# Autodesk Inventor assembly: Frame
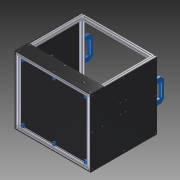
[picture p0: Inventor's stored thumbnail of the model, 180x180]
Saved by Autodesk Inventor 2015 SP1 (Build 190203100, 203)
## iProperties
Created: 2014-08-02
Part Number: Frame
Document SubType Name: Assembly
Designer: Jack
Mass: 9359.12 g
Surface Area: 35492.7 cm^2
Volume: 6557 cm^3
Density: 1.42735 g/cm^3
Author: Jack
Title: Frame
## Documents named in this file (25)
- C:\Users\Jack\ownCloud\Projects\CrossBot\InventorModel\Frame\Frame.iam
- C:\Users\Jack\ownCloud\Projects\CrossBot\InventorModel\Frame\FrameFrontBack.ipt
- C:\Users\Jack\ownCloud\Projects\CrossBot\InventorModel\Frame\FrameSide.ipt
- C:\Users\Jack\ownCloud\Projects\CrossBot\InventorModel\Frame\FrameUpright.ipt
- C:\Users\Jack\ownCloud\Projects\CrossBot\InventorModel\Hardware\Bolts\BlindExtrusionScrew\M5x20BlindScrew.ipt
- C:\Users\Jack\ownCloud\Projects\CrossBot\InventorModel\Frame\FrameExtruderVerticalSupport.ipt
- C:\Users\Jack\ownCloud\Projects\CrossBot\InventorModel\Enclosure\EnclosurePanelBack.ipt
- C:\Users\Jack\ownCloud\Projects\CrossBot\InventorModel\Enclosure\EnclosurePanelBottomFront.ipt
- C:\Users\Jack\ownCloud\Projects\CrossBot\InventorModel\Enclosure\ElectronicsLowerPanel.ipt
- C:\Users\Jack\ownCloud\Projects\CrossBot\InventorModel\Hardware\FrameBrace\FrameBraceHBLFSN5-4.ipt
- C:\Users\Jack\ownCloud\Projects\CrossBot\InventorModel\Enclosure\ElectronicsTopPanel.ipt
- C:\Users\Jack\ownCloud\Projects\CrossBot\InventorModel\Hardware\Bolts\SHCS\SHCS4\SHCS4x10.ipt
- C:\Users\Jack\ownCloud\Projects\CrossBot\InventorModel\Hardware\Nuts\ExtrusionNuts\ExtrusionNutLockHNTR5-4.ipt
- C:\Users\Jack\ownCloud\Projects\CrossBot\InventorModel\Hardware\Bolts\FHS\FHS4\FHS4x10.ipt
- C:\Users\Jack\ownCloud\Projects\CrossBot\InventorModel\Enclosure\EnclosurePanelLeft.ipt
- C:\Users\Jack\ownCloud\Projects\CrossBot\InventorModel\Enclosure\EnclosurePanelRight.ipt
- C:\Users\Jack\ownCloud\Projects\CrossBot\InventorModel\Enclosure\PanelMount.ipt
- C:\Users\Jack\ownCloud\Projects\CrossBot\InventorModel\Hardware\BoltWashers\BoltWasher3\BoltWasher3x18.iam
- C:\Users\Jack\ownCloud\Projects\CrossBot\InventorModel\Hardware\Nuts\Nut3.ipt
- C:\Users\Jack\ownCloud\Projects\CrossBot\InventorModel\Enclosure\PanelLedge.ipt
- C:\Users\Jack\ownCloud\Projects\CrossBot\InventorModel\Hardware\Nuts\ExtrusionNuts\ExtrusionNutHNKK5_4.ipt
- C:\Users\Jack\ownCloud\Projects\CrossBot\InventorModel\Enclosure\SpoolHolder\SpoolHolderSingle.ipt
- C:\Users\Jack\ownCloud\Projects\CrossBot\InventorModel\Hardware\Nuts\Nut4.ipt
- C:\Users\Jack\ownCloud\Projects\CrossBot\InventorModel\Enclosure\FrameHandle.ipt
- C:\Users\Jack\ownCloud\Projects\CrossBot\InventorModel\Hardware\Nuts\ExtrusionNuts\ExtrusionNutHNKK5_5.ipt
## Components (217 placed, 24 different names)
1. FrameSide:6 — Mate:66, Flush:32, Flush:33, Mate:136, Mate:181, Mate:183, Angle:21, Mate:328, Mate:460, Mate:498, Mate:500, Angle:62, Mate:513
2. FrameSide:5 — Mate:64, Flush:28, Flush:30, Mate:138, Mate:180, Mate:184, Angle:36, Angle:51, Mate:398, Mate:497, Mate:499, Angle:63, Mate:512
3. FrameSide:4 — Mate:52, Flush:23, Flush:25, Flush:26, Angle:35, Angle:50, Mate:397, Mate:437, Mate:438
4. FrameSide:3 — Mate:51, Flush:22, Flush:27, Angle:20, Mate:329, Mate:436, Mate:439, Mate:440
5. FrameSide:1 — Mate:1, Flush:1, Flush:2, Mate:3, Flush:5, Flush:6, Mate:18, Mate:22, Angle:25, Mate:342, Flush:114, Mate:363, Angle:95, Angle:96, Mate:616, Mate:617, Flush:165, Mate:618
6. FrameSide:2 — Mate:6, Flush:11, Flush:12, Mate:7, Mate:25, Mate:26, Mate:343, Flush:113, Angle:40, Mate:379, Angle:93, Mate:609, Mate:610, Flush:164, Angle:94, Mate:612
7. FrameExtruderVerticalSupport:1 — Mate:67, Flush:37, Mate:69, Mate:123, Flush:64, Mate:176, Mate:178, Mate:524, Angle:67
8. FrameExtruderVerticalSupport:2 — Mate:68, Flush:36, Mate:70, Mate:124, Flush:65, Mate:177, Mate:179, Mate:522, Angle:68
9. FrameUpright:1 — Mate:1, Flush:1, Flush:2, Mate:2, Flush:3, Flush:4, Mate:42, Mate:43, Mate:48, Mate:49, Mate:53, Flush:21, Flush:22, Mate:61, Mate:62, Mate:65, Mate:66, Flush:33, Flush:34, Mate:70, Flush:69, Mate:132, Mate:191, Mate:199, Angle:22, Angle:23, Angle:24, Mate:325, Mate:326, Mate:327, Angle:47, Angle:48, Angle:49, Mate:390, Mate:391, Mate:392, Mate:523, Angle:69
10. FrameUpright:2 — Mate:3, Flush:5, Flush:6, Mate:5, Flush:9, Flush:10, Mate:12, Mate:13, Mate:19, Mate:21, Mate:36, Mate:37, Mate:50, Mate:51, Mate:54, Mate:55, Mate:56, Flush:61, Mate:137, Flush:71, Mate:192, Mate:193, Mate:281, Angle:17, Angle:18, Mate:323, Angle:19, Mate:324, Angle:26, Angle:27, Mate:338, Mate:339, Flush:115, Mate:517, Angle:65
11. FrameUpright:3 — Mate:7, Mate:8, Flush:13, Mate:38, Mate:39, Mate:46, Mate:47, Mate:52, Flush:23, Flush:24, Mate:57, Mate:58, Mate:63, Mate:64, Flush:28, Flush:29, Mate:139, Flush:72, Mate:194, Mate:195, Angle:28, Angle:29, Mate:336, Mate:337, Flush:116, Mate:365, Angle:32, Mate:367, Mate:369, Angle:33, Angle:34, Mate:515, Angle:64
12. FrameUpright:4 — Mate:4, Flush:7, Flush:8, Mate:6, Flush:11, Flush:12, Mate:40, Mate:41, Mate:44, Mate:45, Mate:59, Mate:60, Mate:69, Mate:134, Flush:70, Mate:190, Mate:198, Mate:373, Angle:37, Mate:375, Angle:38, Mate:377, Angle:39, Flush:135, Mate:381, Angle:41, Angle:43, Angle:44, Mate:395, Mate:396, Mate:525, Angle:66
13. FrameFrontBack:3 — Mate:50, Flush:24, Flush:25, Mate:54, Flush:35, Flush:39, Angle:31, Mate:341, Mate:430, Mate:431, Mate:432, Angle:83, Angle:84, Angle:85, Mate:596, Mate:597, Mate:598, Mate:599
14. FrameFrontBack:6 — Mate:65, Flush:34, Mate:67, Mate:68, Flush:36, Flush:37, Mate:122, Mate:125, Mate:130, Mate:135, Mate:186, Mate:187, Mate:196, Mate:197, Angle:45, Mate:393, Mate:490, Mate:492, Angle:58, Mate:503, Mate:505, Angle:59, Angle:60, Angle:61, Mate:508, Mate:509, Angle:81, Angle:82, Mate:594, Mate:603
15. FrameFrontBack:5 — Mate:63, Flush:29, Flush:30, Flush:32, Flush:35, Mate:73, Mate:182, Mate:185, Angle:30, Mate:340, Mate:447, Flush:138, Mate:488, Mate:489, Angle:86, Angle:87, Angle:88, Mate:600, Mate:604
16. FrameFrontBack:4 — Mate:53, Flush:21, Flush:26, Flush:27, Flush:44, Angle:46, Mate:394, Mate:433, Mate:435, Mate:570, Flush:151, Angle:89, Angle:90, Angle:91, Mate:595, Mate:601, Mate:602
17. FrameFrontBack:1 — Mate:2, Flush:3, Flush:4, Mate:4, Flush:7, Flush:8, Mate:23, Mate:24, Mate:76, Mate:188, Mate:189, Angle:42, Mate:399
18. FrameFrontBack:2 — Mate:5, Flush:9, Flush:10, Mate:8, Flush:13, Flush:20, Mate:20, Mate:27
19. FrameHandle:1 — Mate:610, Flush:164, Mate:611, Mate:613
20. ExtrusionNutHNKK5_5:1 — Angle:93, Mate:609, Mate:611
21. ExtrusionNutHNKK5_5:2 — Angle:94, Mate:612, Mate:613
22. FrameHandle:2 — Flush:165, Mate:618
23. ExtrusionNutHNKK5_5:3 — Angle:95, Mate:616
24. ExtrusionNutHNKK5_5:4 — Angle:96, Mate:617
25. ExtrusionNutHNKK5_4:17 — Mate:583, Angle:89, Mate:602
26. ExtrusionNutHNKK5_4:18 — Mate:584, Angle:90, Mate:601
27. ExtrusionNutHNKK5_4:19 — Mate:585, Angle:91, Mate:595
28. ExtrusionNutHNKK5_4:20 — Mate:586, Angle:85, Mate:596
29. ExtrusionNutHNKK5_4:21 — Mate:587, Angle:84, Mate:598
30. ExtrusionNutHNKK5_4:22 — Mate:588, Angle:83, Mate:599
31. FHS4x10:43 — Mate:576, Flush:155, Mate:583
32. FHS4x10:47 — Mate:572, Flush:156, Mate:584
33. FHS4x10:46 — Mate:573, Flush:157, Mate:585
34. FHS4x10:51 — Mate:581, Flush:162, Mate:587
35. FHS4x10:52 — Mate:582, Flush:163, Mate:588
36. FHS4x10:50 — Mate:580, Flush:161, Mate:586
37. PanelLedge:6 — Mate:570, Flush:151, Mate:571, Mate:572, Flush:156, Flush:158
38. Nut3:1 — Mate:480, Angle:54, Mate:481
39. Nut3:2 — Mate:482, Mate:483, Angle:55
40. Nut3:3 — Mate:478, Mate:479, Angle:53
41. Nut3:4 — Mate:484, Mate:485, Angle:56
42. Nut3:5 — Mate:486, Mate:487, Angle:57
43. BoltWasher3x18:1 [sub-assembly] — Mate:468, Mate:470, Mate:484
44. BoltWasher3x18:2 [sub-assembly] — Mate:464, Mate:472, Mate:480
45. BoltWasher3x18:3 [sub-assembly] — Mate:469, Mate:471, Mate:486
46. BoltWasher3x18:4 [sub-assembly] — Mate:467, Mate:474, Mate:482
47. BoltWasher3x18:5 [sub-assembly] — Mate:466, Mate:475, Mate:478
48. PanelMount:2 — Mate:427, Mate:435, Mate:436, Mate:462, Angle:54, Mate:481, Mate:576, Flush:155
49. PanelMount:4 — Mate:429, Mate:433, Mate:437, Mate:463, Mate:479, Angle:53, Mate:573, Flush:157
50. PanelMount:1 — Mate:425, Mate:430, Mate:438, Mate:483, Angle:55, Mate:580, Flush:161
51. PanelMount:6 — Mate:424, Mate:431, Mate:440, Mate:485, Angle:56, Flush:158, Mate:581, Flush:162
52. PanelMount:5 — Mate:426, Mate:432, Mate:439, Mate:487, Angle:57, Mate:582, Flush:163
53. ElectronicsLowerPanel:1 — Mate:424, Mate:425, Mate:426, Mate:427, Mate:429, Mate:462, Mate:463, Mate:464, Mate:466, Mate:467, Mate:468, Mate:469, Mate:470, Mate:471, Mate:472, Mate:474, Mate:475, Mate:571
54. ExtrusionNutHNKK5_4:23 — Mate:589, Angle:88, Mate:600
55. ExtrusionNutHNKK5_4:24 — Mate:590, Angle:87, Mate:597
56. ExtrusionNutHNKK5_4:25 — Mate:591, Angle:86
57. ExtrusionNutHNKK5_4:26 — Mate:592, Angle:81, Mate:594
58. ExtrusionNutHNKK5_4:27 — Mate:593, Angle:82, Mate:603
59. Nut3:6 — Mate:607, Mate:608, Angle:92
60. BoltWasher3x18:6 [sub-assembly] — Mate:605, Mate:606, Mate:607
61. FHS4x10:45 — Mate:574, Flush:154, Mate:591
62. FHS4x10:44 — Mate:575, Flush:153, Mate:590
63. FHS4x10:42 — Mate:577, Flush:152, Mate:589
64. FHS4x10:49 — Mate:579, Flush:160, Mate:593
65. FHS4x10:48 — Mate:578, Flush:159, Mate:592
66. PanelLedge:1 — Mate:490, Mate:493, Mate:500, Mate:579, Flush:160
67. PanelLedge:3 — Mate:492, Mate:494, Mate:499, Mate:578, Flush:159
68. PanelLedge:4 — Mate:489, Mate:496, Mate:498, Mate:577, Flush:152
69. PanelLedge:5 — Mate:488, Mate:495, Mate:497, Mate:574, Flush:154
70. PanelMount:11 — Mate:447, Mate:451, Mate:460, Mate:501, Mate:575, Flush:153, Mate:605, Mate:608, Angle:92
71. ElectronicsTopPanel:1 — Mate:451, Flush:138, Mate:493, Mate:494, Mate:495, Mate:496, Mate:501, Mate:604, Mate:606
72. ExtrusionNutLockHNTR5-4:1 — Mate:281, Angle:17, Mate:362
73. ExtrusionNutLockHNTR5-4:2 — Mate:315, Angle:18, Mate:323
74. ExtrusionNutLockHNTR5-4:3 — Mate:316, Angle:19, Mate:324
75. ExtrusionNutLockHNTR5-4:4 — Mate:317, Angle:20, Mate:329
76. ExtrusionNutLockHNTR5-4:5 — Mate:318, Angle:21, Mate:328
77. ExtrusionNutLockHNTR5-4:6 — Mate:319, Angle:22, Mate:327
78. ExtrusionNutLockHNTR5-4:7 — Mate:320, Angle:23, Mate:326
79. ExtrusionNutLockHNTR5-4:8 — Mate:321, Angle:24, Mate:325
80. ExtrusionNutLockHNTR5-4:9 — Mate:322, Angle:25, Mate:363
81. FHS4x10:26 — Mate:318, Mate:360, Flush:125
82. FHS4x10:6 — Mate:316, Mate:355, Flush:120
83. FHS4x10:3 — Mate:319, Mate:358, Flush:123
84. FHS4x10:7 — Mate:320, Mate:357, Flush:122
85. FHS4x10:5 — Mate:321, Mate:356, Flush:121
86. FHS4x10:2 — Mate:322, Mate:344, Flush:117
87. FHS4x10:1 — Mate:353, Flush:118, Mate:362
88. FHS4x10:8 — Mate:315, Mate:354, Flush:119
89. FHS4x10:4 — Mate:317, Mate:359, Flush:124
90. EnclosurePanelLeft:1 — Mate:342, Flush:114, Flush:115, Mate:344, Mate:353, Mate:354, Mate:355, Flush:117, Flush:118, Flush:119, Flush:120, Mate:356, Flush:121, Mate:357, Flush:122, Mate:358, Flush:123, Mate:359, Flush:124, Mate:360, Flush:125, Mate:538, Mate:543, Mate:544, Mate:545, Mate:546, Mate:547, Mate:548, Mate:549, Flush:143, Flush:144, Flush:145, Flush:146
91. EnclosurePanelRight:1 — Mate:343, Flush:113, Flush:116, Mate:345, Mate:346, Mate:347, Mate:348, Mate:349, Mate:350, Mate:351, Mate:352, Flush:126, Flush:127, Flush:128, Mate:361, Flush:129, Flush:130, Flush:131, Flush:132, Flush:133, Flush:134, Mate:539, Mate:540, Mate:541, Mate:542, Mate:550, Mate:551, Mate:552, Mate:553, Flush:147, Flush:148, Flush:149, Flush:150
92. ExtrusionNutLockHNTR5-4:16 — Mate:364, Mate:365, Angle:32
93. ExtrusionNutLockHNTR5-4:17 — Mate:366, Mate:367, Angle:34
94. ExtrusionNutLockHNTR5-4:18 — Mate:368, Mate:369, Angle:33
95. ExtrusionNutLockHNTR5-4:19 — Mate:370, Angle:35, Angle:50, Mate:397
96. ExtrusionNutLockHNTR5-4:20 — Mate:371, Angle:36, Angle:51, Mate:398
97. ExtrusionNutLockHNTR5-4:21 — Mate:372, Mate:373, Angle:37
98. ExtrusionNutLockHNTR5-4:22 — Mate:374, Mate:375, Angle:38
99. ExtrusionNutLockHNTR5-4:23 — Mate:376, Mate:377, Angle:39
100. ExtrusionNutLockHNTR5-4:24 — Mate:378, Angle:40, Mate:379
101. FHS4x10:27 — Mate:349, Flush:134, Mate:371
102. FHS4x10:14 — Mate:348, Flush:133, Mate:370
103. FHS4x10:16 — Mate:347, Flush:128, Mate:364
104. FHS4x10:11 — Mate:346, Flush:127, Mate:366
105. FHS4x10:10 — Mate:345, Flush:126, Mate:368
106. FHS4x10:9 — Mate:352, Flush:130, Mate:376
107. FHS4x10:15 — Mate:361, Flush:129, Mate:378
108. FHS4x10:12 — Mate:351, Flush:131, Mate:374
109. FHS4x10:13 — Mate:350, Flush:132, Mate:372
110. EnclosurePanelBack:1 — Mate:76, Flush:44, Mate:298, Mate:299, Mate:300, Mate:301, Mate:302, Mate:303, Mate:304, Mate:305, Flush:96, Flush:97, Flush:98, Flush:99, Flush:100, Flush:101, Flush:102, Flush:103, Mate:306, Flush:104, Flush:135
111. ExtrusionNutLockHNTR5-4:26 — Mate:382, Angle:44, Mate:395
112. ExtrusionNutLockHNTR5-4:27 — Mate:383, Angle:43, Mate:396
113. ExtrusionNutLockHNTR5-4:28 — Mate:384, Angle:42, Mate:399
114. ExtrusionNutLockHNTR5-4:29 — Mate:385, Angle:49, Mate:390
115. ExtrusionNutLockHNTR5-4:30 — Mate:386, Angle:48, Mate:391
116. ExtrusionNutLockHNTR5-4:31 — Mate:387, Angle:47, Mate:392
117. ExtrusionNutLockHNTR5-4:32 — Mate:388, Angle:46, Mate:394
118. ExtrusionNutLockHNTR5-4:33 — Mate:389, Angle:45, Mate:393
119. ExtrusionNutLockHNTR5-4:25 — Mate:380, Mate:381, Angle:41
120. FHS4x10:22 — Mate:303, Flush:98, Mate:383
121. FHS4x10:25 — Mate:306, Flush:104, Mate:384
122. FHS4x10:23 — Mate:304, Flush:97, Mate:382
123. FHS4x10:24 — Mate:305, Flush:96, Mate:380
124. FHS4x10:21 — Mate:302, Flush:99, Mate:389
125. FHS4x10:20 — Mate:301, Flush:100, Mate:388
126. FHS4x10:19 — Mate:300, Flush:101, Mate:387
127. FHS4x10:18 — Mate:299, Flush:102, Mate:386
128. FHS4x10:17 — Mate:298, Flush:103, Mate:385
129. EnclosurePanelBottomFront:1 — Mate:73, Flush:39, Flush:61, Mate:309, Flush:107, Mate:310, Flush:108, Mate:311, Flush:109, Mate:312, Flush:110, Mate:313, Mate:314, Flush:111, Flush:112
130. ExtrusionNutLockHNTR5-4:10 — Mate:330, Angle:27, Mate:338
131. ExtrusionNutLockHNTR5-4:11 — Mate:331, Angle:26, Mate:339
132. ExtrusionNutLockHNTR5-4:12 — Mate:332, Angle:31, Mate:341
133. ExtrusionNutLockHNTR5-4:13 — Mate:333, Angle:30, Mate:340
134. ExtrusionNutLockHNTR5-4:14 — Mate:334, Angle:28, Mate:336
135. ExtrusionNutLockHNTR5-4:15 — Mate:335, Angle:29, Mate:337
136. FHS4x10:28 — Mate:309, Flush:107, Mate:331
137. FHS4x10:29 — Mate:310, Flush:108, Mate:330
138. FHS4x10:30 — Mate:311, Flush:109, Mate:332
139. FHS4x10:31 — Mate:312, Flush:110, Mate:333
140. FHS4x10:32 — Mate:313, Flush:112, Mate:335
141. FHS4x10:33 — Mate:314, Flush:111, Mate:334
142. M5x20BlindScrew:17 — Mate:176, Mate:189
143. M5x20BlindScrew:18 — Mate:177, Mate:188
144. M5x20BlindScrew:19 — Mate:178, Mate:187
145. M5x20BlindScrew:20 — Mate:179, Mate:186
146. M5x20BlindScrew:21 — Mate:180, Mate:190
147. M5x20BlindScrew:22 — Mate:181, Mate:191
148. M5x20BlindScrew:23 — Mate:182, Mate:192
149. M5x20BlindScrew:24 — Mate:183, Mate:193
150. M5x20BlindScrew:25 — Mate:184, Mate:194
151. M5x20BlindScrew:26 — Mate:185, Mate:195
152. M5x20BlindScrew:27 — Mate:196, Mate:199
153. M5x20BlindScrew:28 — Mate:197, Mate:198
154. M5x20BlindScrew:1 — Mate:22, Mate:43
155. M5x20BlindScrew:2 — Mate:24, Mate:40
156. M5x20BlindScrew:3 — Mate:49, Mate:61
157. M5x20BlindScrew:4 — Mate:36, Mate:55
158. M5x20BlindScrew:5 — Mate:48, Mate:62
159. M5x20BlindScrew:6 — Mate:44, Mate:60
160. M5x20BlindScrew:7 — Mate:46, Mate:58
161. M5x20BlindScrew:8 — Mate:27, Mate:38
162. M5x20BlindScrew:9 — Mate:26, Mate:39
163. M5x20BlindScrew:10 — Mate:25, Mate:41
164. M5x20BlindScrew:11 — Mate:20, Mate:21
165. M5x20BlindScrew:12 — Mate:23, Mate:42
166. M5x20BlindScrew:13 — Mate:37, Mate:56
167. M5x20BlindScrew:14 — Mate:45, Mate:59
168. M5x20BlindScrew:15 — Mate:47, Mate:57
169. M5x20BlindScrew:16 — Mate:18, Mate:19
170. ExtrusionNutHNKK5_4:1 — Mate:502, Angle:58, Mate:503
171. ExtrusionNutHNKK5_4:2 — Mate:504, Mate:505, Angle:59
172. ExtrusionNutHNKK5_4:3 — Mate:506, Angle:60, Mate:509
173. ExtrusionNutHNKK5_4:4 — Mate:507, Angle:61, Mate:508
174. ExtrusionNutHNKK5_4:5 — Mate:511, Angle:62, Mate:513
175. ExtrusionNutHNKK5_4:6 — Mate:510, Angle:63, Mate:512
176. ExtrusionNutHNKK5_4:7 — Mate:514, Mate:515, Angle:64
177. ExtrusionNutHNKK5_4:8 — Mate:516, Mate:517, Angle:65
178. ExtrusionNutHNKK5_4:9 — Mate:518, Mate:525, Angle:66
179. ExtrusionNutHNKK5_4:10 — Mate:519, Mate:524, Angle:67
180. ExtrusionNutHNKK5_4:11 — Mate:521, Mate:522, Angle:68
181. ExtrusionNutHNKK5_4:12 — Mate:520, Mate:523, Angle:69
182. SHCS4x10:3 — Mate:201, Mate:202, Mate:516
183. SHCS4x10:12 — Mate:200, Mate:203, Mate:511
184. SHCS4x10:9 — Mate:232, Mate:244, Mate:520
185. SHCS4x10:11 — Mate:233, Mate:247, Mate:507
186. SHCS4x10:6 — Mate:235, Mate:243, Mate:521
187. SHCS4x10:8 — Mate:234, Mate:246, Mate:502
188. SHCS4x10:7 — Mate:236, Mate:245, Mate:504
189. SHCS4x10:1 — Mate:237, Mate:242, Mate:519
190. SHCS4x10:2 — Mate:238, Mate:241, Mate:506
191. SHCS4x10:5 — Mate:239, Mate:240, Mate:518
192. SHCS4x10:4 — Mate:205, Mate:206, Mate:514
193. SHCS4x10:10 — Mate:204, Mate:207, Mate:510
194. FrameBraceHBLFSN5-4:1 — Mate:122, Mate:123, Flush:64, Mate:236, Mate:237, Mate:242, Mate:245
195. FrameBraceHBLFSN5-4:2 — Mate:124, Flush:65, Mate:125, Mate:234, Mate:235, Mate:243, Mate:246
196. FrameBraceHBLFSN5-4:5 — Mate:130, Flush:69, Mate:132, Mate:232, Mate:233, Mate:244, Mate:247
197. FrameBraceHBLFSN5-4:7 — Mate:134, Mate:135, Flush:70, Mate:238, Mate:239, Mate:240, Mate:241
198. FrameBraceHBLFSN5-4:8 — Mate:136, Mate:137, Flush:71, Mate:200, Mate:201, Mate:202, Mate:203
199. FrameBraceHBLFSN5-4:9 — Mate:138, Mate:139, Flush:72, Mate:204, Mate:205, Mate:206, Mate:207
200. Nut4:1 — Mate:558, Mate:566, Angle:79
201. Nut4:3 — Mate:559, Mate:567, Angle:80
202. Nut4:6 — Mate:560, Mate:568, Angle:78
203. Nut4:8 — Mate:561, Mate:569, Angle:77
204. FHS4x10:38 — Mate:547, Flush:145, Mate:558
205. FHS4x10:40 — Mate:546, Flush:146, Mate:559
206. SpoolHolderSingle:1 — Mate:538, Mate:543, Mate:544, Mate:545, Mate:566, Mate:567, Mate:568, Mate:569, Angle:77, Angle:78, Angle:79, Angle:80
207. FHS4x10:34 — Mate:548, Flush:144, Mate:560
208. FHS4x10:35 — Mate:549, Flush:143, Mate:561
209. Nut4:2 — Mate:554, Mate:562, Angle:75
210. Nut4:4 — Mate:555, Mate:564, Angle:74
211. Nut4:5 — Mate:557, Mate:565, Angle:73
212. Nut4:7 — Mate:556, Mate:563, Angle:76
213. FHS4x10:41 — Mate:552, Flush:148, Mate:554
214. FHS4x10:36 — Mate:550, Flush:150, Mate:556
215. FHS4x10:39 — Mate:553, Flush:147, Mate:555
216. FHS4x10:37 — Mate:551, Flush:149, Mate:557
217. SpoolHolderSingle:2 — Mate:539, Mate:540, Mate:541, Mate:542, Mate:562, Mate:563, Mate:564, Mate:565, Angle:73, Angle:74, Angle:75, Angle:76
## Relationships (554: Mate 376, Flush 102, Angle 76)
- Mate:1: FrameSide:1 ↔ FrameUpright:1
- Flush:1: FrameSide:1 ↔ FrameUpright:1
- Flush:2: FrameSide:1 ↔ FrameUpright:1
- Mate:2: FrameUpright:1 ↔ FrameFrontBack:1
- Flush:3: FrameUpright:1 ↔ FrameFrontBack:1
- Flush:4: FrameUpright:1 ↔ FrameFrontBack:1
- Mate:3: FrameSide:1 ↔ FrameUpright:2
- Flush:5: FrameSide:1 ↔ FrameUpright:2
- Flush:6: FrameSide:1 ↔ FrameUpright:2
- Mate:4: FrameUpright:4 ↔ FrameFrontBack:1
- Flush:7: FrameUpright:4 ↔ FrameFrontBack:1
- Flush:8: FrameUpright:4 ↔ FrameFrontBack:1
- Mate:5: FrameUpright:2 ↔ FrameFrontBack:2
- Flush:9: FrameUpright:2 ↔ FrameFrontBack:2
- Flush:10: FrameUpright:2 ↔ FrameFrontBack:2
- Mate:6: FrameSide:2 ↔ FrameUpright:4
- Flush:11: FrameSide:2 ↔ FrameUpright:4
- Flush:12: FrameSide:2 ↔ FrameUpright:4
- Mate:7: FrameSide:2 ↔ FrameUpright:3
- Mate:8: FrameUpright:3 ↔ FrameFrontBack:2
- Flush:13: FrameUpright:3 ↔ FrameFrontBack:2
- Mate:12: FrameUpright:2
- Mate:13: FrameUpright:2
- Flush:20: FrameFrontBack:2
- Mate:18: FrameSide:1 ↔ M5x20BlindScrew:16
- Mate:19: FrameUpright:2 ↔ M5x20BlindScrew:16
- Mate:20: FrameFrontBack:2 ↔ M5x20BlindScrew:11
- Mate:21: FrameUpright:2 ↔ M5x20BlindScrew:11
- Mate:22: FrameSide:1 ↔ M5x20BlindScrew:1
- Mate:23: FrameFrontBack:1 ↔ M5x20BlindScrew:12
- Mate:24: FrameFrontBack:1 ↔ M5x20BlindScrew:2
- Mate:25: FrameSide:2 ↔ M5x20BlindScrew:10
- Mate:26: FrameSide:2 ↔ M5x20BlindScrew:9
- Mate:27: FrameFrontBack:2 ↔ M5x20BlindScrew:8
- Mate:36: FrameUpright:2 ↔ M5x20BlindScrew:4
- Mate:37: FrameUpright:2 ↔ M5x20BlindScrew:13
- Mate:38: FrameUpright:3 ↔ M5x20BlindScrew:8
- Mate:39: FrameUpright:3 ↔ M5x20BlindScrew:9
- Mate:40: FrameUpright:4 ↔ M5x20BlindScrew:2
- Mate:41: FrameUpright:4 ↔ M5x20BlindScrew:10
- Mate:42: FrameUpright:1 ↔ M5x20BlindScrew:12
- Mate:43: FrameUpright:1 ↔ M5x20BlindScrew:1
- Mate:44: FrameUpright:4 ↔ M5x20BlindScrew:6
- Mate:45: FrameUpright:4 ↔ M5x20BlindScrew:14
- Mate:46: FrameUpright:3 ↔ M5x20BlindScrew:7
- Mate:47: FrameUpright:3 ↔ M5x20BlindScrew:15
- Mate:48: FrameUpright:1 ↔ M5x20BlindScrew:5
- Mate:49: FrameUpright:1 ↔ M5x20BlindScrew:3
- Mate:50: FrameUpright:2 ↔ FrameFrontBack:3
- Mate:51: FrameSide:3 ↔ FrameUpright:2
- Mate:52: FrameSide:4 ↔ FrameUpright:3
- Mate:53: FrameUpright:1 ↔ FrameFrontBack:4
- Flush:21: FrameUpright:1 ↔ FrameFrontBack:4
- Flush:22: FrameSide:3 ↔ FrameUpright:1
- Flush:23: FrameSide:4 ↔ FrameUpright:3
- Flush:24: FrameUpright:3 ↔ FrameFrontBack:3
- Flush:25: FrameSide:4 ↔ FrameFrontBack:3
- Flush:26: FrameSide:4 ↔ FrameFrontBack:4
- Flush:27: FrameSide:3 ↔ FrameFrontBack:4
- Mate:54 (-20 mm): FrameUpright:2 ↔ FrameFrontBack:3
- Mate:55: FrameUpright:2 ↔ M5x20BlindScrew:4
- Mate:56: FrameUpright:2 ↔ M5x20BlindScrew:13
- Mate:57: FrameUpright:3 ↔ M5x20BlindScrew:15
- Mate:58: FrameUpright:3 ↔ M5x20BlindScrew:7
- Mate:59: FrameUpright:4 ↔ M5x20BlindScrew:14
- Mate:60: FrameUpright:4 ↔ M5x20BlindScrew:6
- Mate:61: FrameUpright:1 ↔ M5x20BlindScrew:3
- Mate:62: FrameUpright:1 ↔ M5x20BlindScrew:5
- Mate:63: FrameUpright:3 ↔ FrameFrontBack:5
- Mate:64: FrameSide:5 ↔ FrameUpright:3
- Flush:28: FrameSide:5 ↔ FrameUpright:3
- Flush:29: FrameUpright:3 ↔ FrameFrontBack:5
- Flush:30: FrameSide:5 ↔ FrameFrontBack:5
- [Flush]: FrameSide:6 ↔ FrameFrontBack:6
- Mate:65: FrameUpright:1 ↔ FrameFrontBack:6
- Mate:66: FrameSide:6 ↔ FrameUpright:1
- Flush:32: FrameSide:6 ↔ FrameFrontBack:5
- Flush:33: FrameSide:6 ↔ FrameUpright:1
- Flush:34: FrameUpright:1 ↔ FrameFrontBack:6
- Flush:35 (-65 mm): FrameFrontBack:3 ↔ FrameFrontBack:5
- Mate:67: FrameExtruderVerticalSupport:1 ↔ FrameFrontBack:6
- Mate:68: FrameExtruderVerticalSupport:2 ↔ FrameFrontBack:6
- Flush:36: FrameExtruderVerticalSupport:2 ↔ FrameFrontBack:6
- Flush:37: FrameExtruderVerticalSupport:1 ↔ FrameFrontBack:6
- Mate:69 (88 mm): FrameExtruderVerticalSupport:1 ↔ FrameUpright:4
- Mate:70 (88 mm): FrameExtruderVerticalSupport:2 ↔ FrameUpright:1
- Mate:73: FrameFrontBack:5 ↔ EnclosurePanelBottomFront:1
- Flush:39: FrameFrontBack:3 ↔ EnclosurePanelBottomFront:1
- Mate:76: FrameFrontBack:1 ↔ EnclosurePanelBack:1
- Flush:44: FrameFrontBack:4 ↔ EnclosurePanelBack:1
- Flush:61 (-4.7625 mm): FrameUpright:2 ↔ EnclosurePanelBottomFront:1
- Mate:122: FrameFrontBack:6 ↔ FrameBraceHBLFSN5-4:1
- Mate:123: FrameExtruderVerticalSupport:1 ↔ FrameBraceHBLFSN5-4:1
- Flush:64: FrameExtruderVerticalSupport:1 ↔ FrameBraceHBLFSN5-4:1
- Mate:124: FrameExtruderVerticalSupport:2 ↔ FrameBraceHBLFSN5-4:2
- Flush:65: FrameExtruderVerticalSupport:2 ↔ FrameBraceHBLFSN5-4:2
- Mate:125: FrameFrontBack:6 ↔ FrameBraceHBLFSN5-4:2
- Mate:130: FrameFrontBack:6 ↔ FrameBraceHBLFSN5-4:5
- Flush:69: FrameUpright:1 ↔ FrameBraceHBLFSN5-4:5
- Mate:132: FrameUpright:1 ↔ FrameBraceHBLFSN5-4:5
- Mate:134: FrameUpright:4 ↔ FrameBraceHBLFSN5-4:7
- Mate:135: FrameFrontBack:6 ↔ FrameBraceHBLFSN5-4:7
- Flush:70: FrameUpright:4 ↔ FrameBraceHBLFSN5-4:7
- Mate:136: FrameSide:6 ↔ FrameBraceHBLFSN5-4:8
- Mate:137: FrameUpright:2 ↔ FrameBraceHBLFSN5-4:8
- Flush:71: FrameUpright:2 ↔ FrameBraceHBLFSN5-4:8
- Mate:138: FrameSide:5 ↔ FrameBraceHBLFSN5-4:9
- Mate:139: FrameUpright:3 ↔ FrameBraceHBLFSN5-4:9
- Flush:72: FrameUpright:3 ↔ FrameBraceHBLFSN5-4:9
- Mate:176: FrameExtruderVerticalSupport:1 ↔ M5x20BlindScrew:17
- Mate:177: FrameExtruderVerticalSupport:2 ↔ M5x20BlindScrew:18
- Mate:178: FrameExtruderVerticalSupport:1 ↔ M5x20BlindScrew:19
- Mate:179: FrameExtruderVerticalSupport:2 ↔ M5x20BlindScrew:20
- Mate:180: FrameSide:5 ↔ M5x20BlindScrew:21
- Mate:181: FrameSide:6 ↔ M5x20BlindScrew:22
- Mate:182: FrameFrontBack:5 ↔ M5x20BlindScrew:23
- Mate:183: FrameSide:6 ↔ M5x20BlindScrew:24
- Mate:184: FrameSide:5 ↔ M5x20BlindScrew:25
- Mate:185: FrameFrontBack:5 ↔ M5x20BlindScrew:26
- Mate:186: FrameFrontBack:6 ↔ M5x20BlindScrew:20
- Mate:187: FrameFrontBack:6 ↔ M5x20BlindScrew:19
- Mate:188: FrameFrontBack:1 ↔ M5x20BlindScrew:18
- Mate:189: FrameFrontBack:1 ↔ M5x20BlindScrew:17
- Mate:190: FrameUpright:4 ↔ M5x20BlindScrew:21
- Mate:191: FrameUpright:1 ↔ M5x20BlindScrew:22
- Mate:192: FrameUpright:2 ↔ M5x20BlindScrew:23
- Mate:193: FrameUpright:2 ↔ M5x20BlindScrew:24
- Mate:194: FrameUpright:3 ↔ M5x20BlindScrew:25
- Mate:195: FrameUpright:3 ↔ M5x20BlindScrew:26
- Mate:196: FrameFrontBack:6 ↔ M5x20BlindScrew:27
- Mate:197: FrameFrontBack:6 ↔ M5x20BlindScrew:28
- Mate:198: FrameUpright:4 ↔ M5x20BlindScrew:28
- Mate:199: FrameUpright:1 ↔ M5x20BlindScrew:27
- Mate:200: SHCS4x10:12 ↔ FrameBraceHBLFSN5-4:8
- Mate:201: SHCS4x10:3 ↔ FrameBraceHBLFSN5-4:8
- Mate:202: SHCS4x10:3 ↔ FrameBraceHBLFSN5-4:8
- Mate:203: SHCS4x10:12 ↔ FrameBraceHBLFSN5-4:8
- Mate:204: SHCS4x10:10 ↔ FrameBraceHBLFSN5-4:9
- Mate:205: SHCS4x10:4 ↔ FrameBraceHBLFSN5-4:9
- Mate:206: SHCS4x10:4 ↔ FrameBraceHBLFSN5-4:9
- Mate:207: SHCS4x10:10 ↔ FrameBraceHBLFSN5-4:9
- Mate:232: SHCS4x10:9 ↔ FrameBraceHBLFSN5-4:5
- Mate:233: SHCS4x10:11 ↔ FrameBraceHBLFSN5-4:5
- Mate:234: SHCS4x10:8 ↔ FrameBraceHBLFSN5-4:2
- Mate:235: SHCS4x10:6 ↔ FrameBraceHBLFSN5-4:2
- Mate:236: SHCS4x10:7 ↔ FrameBraceHBLFSN5-4:1
- Mate:237: SHCS4x10:1 ↔ FrameBraceHBLFSN5-4:1
- Mate:238: SHCS4x10:2 ↔ FrameBraceHBLFSN5-4:7
- Mate:239: SHCS4x10:5 ↔ FrameBraceHBLFSN5-4:7
- Mate:240: SHCS4x10:5 ↔ FrameBraceHBLFSN5-4:7
- Mate:241: SHCS4x10:2 ↔ FrameBraceHBLFSN5-4:7
- Mate:242: SHCS4x10:1 ↔ FrameBraceHBLFSN5-4:1
- Mate:243: SHCS4x10:6 ↔ FrameBraceHBLFSN5-4:2
- Mate:244: SHCS4x10:9 ↔ FrameBraceHBLFSN5-4:5
- Mate:245: SHCS4x10:7 ↔ FrameBraceHBLFSN5-4:1
- Mate:246: SHCS4x10:8 ↔ FrameBraceHBLFSN5-4:2
- Mate:247: SHCS4x10:11 ↔ FrameBraceHBLFSN5-4:5
- Mate:281: FrameUpright:2 ↔ ExtrusionNutLockHNTR5-4:1
- Angle:17 (180 deg): FrameUpright:2 ↔ ExtrusionNutLockHNTR5-4:1
- Mate:298: EnclosurePanelBack:1 ↔ FHS4x10:17
- Mate:299: EnclosurePanelBack:1 ↔ FHS4x10:18
- Mate:300: EnclosurePanelBack:1 ↔ FHS4x10:19
- Mate:301: EnclosurePanelBack:1 ↔ FHS4x10:20
- Mate:302: EnclosurePanelBack:1 ↔ FHS4x10:21
- Mate:303: EnclosurePanelBack:1 ↔ FHS4x10:22
- Mate:304: EnclosurePanelBack:1 ↔ FHS4x10:23
- Mate:305: EnclosurePanelBack:1 ↔ FHS4x10:24
- Flush:96: EnclosurePanelBack:1 ↔ FHS4x10:24
- Flush:97: EnclosurePanelBack:1 ↔ FHS4x10:23
- Flush:98: EnclosurePanelBack:1 ↔ FHS4x10:22
- Flush:99: EnclosurePanelBack:1 ↔ FHS4x10:21
- Flush:100: EnclosurePanelBack:1 ↔ FHS4x10:20
- Flush:101: EnclosurePanelBack:1 ↔ FHS4x10:19
- Flush:102: EnclosurePanelBack:1 ↔ FHS4x10:18
- Flush:103: EnclosurePanelBack:1 ↔ FHS4x10:17
- Mate:306: EnclosurePanelBack:1 ↔ FHS4x10:25
- Flush:104: EnclosurePanelBack:1 ↔ FHS4x10:25
- Mate:309: EnclosurePanelBottomFront:1 ↔ FHS4x10:28
- Flush:107: EnclosurePanelBottomFront:1 ↔ FHS4x10:28
- Mate:310: EnclosurePanelBottomFront:1 ↔ FHS4x10:29
- Flush:108: EnclosurePanelBottomFront:1 ↔ FHS4x10:29
- Mate:311: EnclosurePanelBottomFront:1 ↔ FHS4x10:30
- Flush:109: EnclosurePanelBottomFront:1 ↔ FHS4x10:30
- Mate:312: EnclosurePanelBottomFront:1 ↔ FHS4x10:31
- Flush:110: EnclosurePanelBottomFront:1 ↔ FHS4x10:31
- Mate:313: EnclosurePanelBottomFront:1 ↔ FHS4x10:32
- Mate:314: EnclosurePanelBottomFront:1 ↔ FHS4x10:33
- Flush:111: EnclosurePanelBottomFront:1 ↔ FHS4x10:33
- Flush:112: EnclosurePanelBottomFront:1 ↔ FHS4x10:32
- Mate:315: ExtrusionNutLockHNTR5-4:2 ↔ FHS4x10:8
- Mate:316: ExtrusionNutLockHNTR5-4:3 ↔ FHS4x10:6
- Mate:317: ExtrusionNutLockHNTR5-4:4 ↔ FHS4x10:4
- Mate:318: ExtrusionNutLockHNTR5-4:5 ↔ FHS4x10:26
- Mate:319: ExtrusionNutLockHNTR5-4:6 ↔ FHS4x10:3
- Mate:320: ExtrusionNutLockHNTR5-4:7 ↔ FHS4x10:7
- Mate:321: ExtrusionNutLockHNTR5-4:8 ↔ FHS4x10:5
- Mate:322: ExtrusionNutLockHNTR5-4:9 ↔ FHS4x10:2
- Angle:18 (180 deg): FrameUpright:2 ↔ ExtrusionNutLockHNTR5-4:2
- Mate:323: FrameUpright:2 ↔ ExtrusionNutLockHNTR5-4:2
- Angle:19 (0 deg): FrameUpright:2 ↔ ExtrusionNutLockHNTR5-4:3
- Mate:324: FrameUpright:2 ↔ ExtrusionNutLockHNTR5-4:3
- Angle:20 (0 deg): FrameSide:3 ↔ ExtrusionNutLockHNTR5-4:4
- Angle:21 (0 deg): FrameSide:6 ↔ ExtrusionNutLockHNTR5-4:5
- Angle:22 (0 deg): FrameUpright:1 ↔ ExtrusionNutLockHNTR5-4:6
- Angle:23 (0 deg): FrameUpright:1 ↔ ExtrusionNutLockHNTR5-4:7
- Angle:24 (0 deg): FrameUpright:1 ↔ ExtrusionNutLockHNTR5-4:8
- Angle:25 (0 deg): FrameSide:1 ↔ ExtrusionNutLockHNTR5-4:9
- Mate:325: FrameUpright:1 ↔ ExtrusionNutLockHNTR5-4:8
- Mate:326: FrameUpright:1 ↔ ExtrusionNutLockHNTR5-4:7
- Mate:327: FrameUpright:1 ↔ ExtrusionNutLockHNTR5-4:6
- Mate:328: FrameSide:6 ↔ ExtrusionNutLockHNTR5-4:5
- Mate:329: FrameSide:3 ↔ ExtrusionNutLockHNTR5-4:4
- Mate:330: ExtrusionNutLockHNTR5-4:10 ↔ FHS4x10:29
- Mate:331: ExtrusionNutLockHNTR5-4:11 ↔ FHS4x10:28
- Mate:332: ExtrusionNutLockHNTR5-4:12 ↔ FHS4x10:30
- Mate:333: ExtrusionNutLockHNTR5-4:13 ↔ FHS4x10:31
- Mate:334: ExtrusionNutLockHNTR5-4:14 ↔ FHS4x10:33
- Mate:335: ExtrusionNutLockHNTR5-4:15 ↔ FHS4x10:32
- Angle:26 (180 deg): FrameUpright:2 ↔ ExtrusionNutLockHNTR5-4:11
- Angle:27 (180 deg): FrameUpright:2 ↔ ExtrusionNutLockHNTR5-4:10
- Angle:28 (180 deg): FrameUpright:3 ↔ ExtrusionNutLockHNTR5-4:14
- Angle:29 (0 deg): FrameUpright:3 ↔ ExtrusionNutLockHNTR5-4:15
- Angle:30 (0 deg): FrameFrontBack:5 ↔ ExtrusionNutLockHNTR5-4:13
- Angle:31 (0 deg): FrameFrontBack:3 ↔ ExtrusionNutLockHNTR5-4:12
- Mate:336: FrameUpright:3 ↔ ExtrusionNutLockHNTR5-4:14
- Mate:337: FrameUpright:3 ↔ ExtrusionNutLockHNTR5-4:15
- Mate:338: FrameUpright:2 ↔ ExtrusionNutLockHNTR5-4:10
- Mate:339: FrameUpright:2 ↔ ExtrusionNutLockHNTR5-4:11
- Mate:340: FrameFrontBack:5 ↔ ExtrusionNutLockHNTR5-4:13
- Mate:341: FrameFrontBack:3 ↔ ExtrusionNutLockHNTR5-4:12
- Mate:342: FrameSide:1 ↔ EnclosurePanelLeft:1
- Mate:343: FrameSide:2 ↔ EnclosurePanelRight:1
- Flush:113: FrameSide:2 ↔ EnclosurePanelRight:1
- Flush:114: FrameSide:1 ↔ EnclosurePanelLeft:1
- Flush:115: FrameUpright:2 ↔ EnclosurePanelLeft:1
- Flush:116: FrameUpright:3 ↔ EnclosurePanelRight:1
- Mate:344: FHS4x10:2 ↔ EnclosurePanelLeft:1
- Mate:345: EnclosurePanelRight:1 ↔ FHS4x10:10
- Mate:346: EnclosurePanelRight:1 ↔ FHS4x10:11
- Mate:347: EnclosurePanelRight:1 ↔ FHS4x10:16
- Mate:348: EnclosurePanelRight:1 ↔ FHS4x10:14
- Mate:349: EnclosurePanelRight:1 ↔ FHS4x10:27
- Mate:350: EnclosurePanelRight:1 ↔ FHS4x10:13
- Mate:351: EnclosurePanelRight:1 ↔ FHS4x10:12
- Mate:352: EnclosurePanelRight:1 ↔ FHS4x10:9
- Mate:353: FHS4x10:1 ↔ EnclosurePanelLeft:1
- Mate:354: FHS4x10:8 ↔ EnclosurePanelLeft:1
- Mate:355: FHS4x10:6 ↔ EnclosurePanelLeft:1
- Flush:117: FHS4x10:2 ↔ EnclosurePanelLeft:1
- Flush:118: FHS4x10:1 ↔ EnclosurePanelLeft:1
- Flush:119: FHS4x10:8 ↔ EnclosurePanelLeft:1
- Flush:120: FHS4x10:6 ↔ EnclosurePanelLeft:1
- Mate:356: FHS4x10:5 ↔ EnclosurePanelLeft:1
- Flush:121: FHS4x10:5 ↔ EnclosurePanelLeft:1
- Mate:357: FHS4x10:7 ↔ EnclosurePanelLeft:1
- Flush:122: FHS4x10:7 ↔ EnclosurePanelLeft:1
- Mate:358: FHS4x10:3 ↔ EnclosurePanelLeft:1
- Flush:123: FHS4x10:3 ↔ EnclosurePanelLeft:1
- Mate:359: FHS4x10:4 ↔ EnclosurePanelLeft:1
- Flush:124: FHS4x10:4 ↔ EnclosurePanelLeft:1
- Mate:360: FHS4x10:26 ↔ EnclosurePanelLeft:1
- Flush:125: FHS4x10:26 ↔ EnclosurePanelLeft:1
- Flush:126: EnclosurePanelRight:1 ↔ FHS4x10:10
- Flush:127: EnclosurePanelRight:1 ↔ FHS4x10:11
- Flush:128: EnclosurePanelRight:1 ↔ FHS4x10:16
- Mate:361: EnclosurePanelRight:1 ↔ FHS4x10:15
- Flush:129: EnclosurePanelRight:1 ↔ FHS4x10:15
- Flush:130: EnclosurePanelRight:1 ↔ FHS4x10:9
- Flush:131: EnclosurePanelRight:1 ↔ FHS4x10:12
- Flush:132: EnclosurePanelRight:1 ↔ FHS4x10:13
- Flush:133: EnclosurePanelRight:1 ↔ FHS4x10:14
- Flush:134: EnclosurePanelRight:1 ↔ FHS4x10:27
- Mate:362: ExtrusionNutLockHNTR5-4:1 ↔ FHS4x10:1
- Mate:363: FrameSide:1 ↔ ExtrusionNutLockHNTR5-4:9
- Mate:364: ExtrusionNutLockHNTR5-4:16 ↔ FHS4x10:16
- Mate:365: FrameUpright:3 ↔ ExtrusionNutLockHNTR5-4:16
- Angle:32 (0 deg): FrameUpright:3 ↔ ExtrusionNutLockHNTR5-4:16
- Mate:366: ExtrusionNutLockHNTR5-4:17 ↔ FHS4x10:11
- Mate:367: FrameUpright:3 ↔ ExtrusionNutLockHNTR5-4:17
- Mate:368: ExtrusionNutLockHNTR5-4:18 ↔ FHS4x10:10
- Mate:369: FrameUpright:3 ↔ ExtrusionNutLockHNTR5-4:18
- Angle:33 (180 deg): FrameUpright:3 ↔ ExtrusionNutLockHNTR5-4:18
- Angle:34 (0 deg): FrameUpright:3 ↔ ExtrusionNutLockHNTR5-4:17
- Mate:370: ExtrusionNutLockHNTR5-4:19 ↔ FHS4x10:14
- Angle:35 (0 deg): FrameSide:4 ↔ ExtrusionNutLockHNTR5-4:19
- Mate:371: ExtrusionNutLockHNTR5-4:20 ↔ FHS4x10:27
- Angle:36 (0 deg): FrameSide:5 ↔ ExtrusionNutLockHNTR5-4:20
- Mate:372: ExtrusionNutLockHNTR5-4:21 ↔ FHS4x10:13
- Mate:373: FrameUpright:4 ↔ ExtrusionNutLockHNTR5-4:21
- Angle:37 (0 deg): FrameUpright:4 ↔ ExtrusionNutLockHNTR5-4:21
- Mate:374: ExtrusionNutLockHNTR5-4:22 ↔ FHS4x10:12
- Mate:375: FrameUpright:4 ↔ ExtrusionNutLockHNTR5-4:22
- Angle:38 (0 deg): FrameUpright:4 ↔ ExtrusionNutLockHNTR5-4:22
- Mate:376: ExtrusionNutLockHNTR5-4:23 ↔ FHS4x10:9
- Mate:377: FrameUpright:4 ↔ ExtrusionNutLockHNTR5-4:23
- Angle:39 (0 deg): FrameUpright:4 ↔ ExtrusionNutLockHNTR5-4:23
- Mate:378: ExtrusionNutLockHNTR5-4:24 ↔ FHS4x10:15
- Angle:40 (0 deg): FrameSide:2 ↔ ExtrusionNutLockHNTR5-4:24
- Mate:379: FrameSide:2 ↔ ExtrusionNutLockHNTR5-4:24
- Mate:380: ExtrusionNutLockHNTR5-4:25 ↔ FHS4x10:24
- Flush:135: FrameUpright:4 ↔ EnclosurePanelBack:1
- Mate:381: FrameUpright:4 ↔ ExtrusionNutLockHNTR5-4:25
- Angle:41 (0 deg): FrameUpright:4 ↔ ExtrusionNutLockHNTR5-4:25
- Mate:382: ExtrusionNutLockHNTR5-4:26 ↔ FHS4x10:23
- Mate:383: ExtrusionNutLockHNTR5-4:27 ↔ FHS4x10:22
- Mate:384: ExtrusionNutLockHNTR5-4:28 ↔ FHS4x10:25
- Mate:385: ExtrusionNutLockHNTR5-4:29 ↔ FHS4x10:17
- Mate:386: ExtrusionNutLockHNTR5-4:30 ↔ FHS4x10:18
- Mate:387: ExtrusionNutLockHNTR5-4:31 ↔ FHS4x10:19
- Mate:388: ExtrusionNutLockHNTR5-4:32 ↔ FHS4x10:20
- Mate:389: ExtrusionNutLockHNTR5-4:33 ↔ FHS4x10:21
- Angle:42 (0 deg): FrameFrontBack:1 ↔ ExtrusionNutLockHNTR5-4:28
- Angle:43 (0 deg): FrameUpright:4 ↔ ExtrusionNutLockHNTR5-4:27
- Angle:44 (0 deg): FrameUpright:4 ↔ ExtrusionNutLockHNTR5-4:26
- Angle:45 (0 deg): FrameFrontBack:6 ↔ ExtrusionNutLockHNTR5-4:33
- Angle:46 (0 deg): FrameFrontBack:4 ↔ ExtrusionNutLockHNTR5-4:32
- Angle:47 (0 deg): FrameUpright:1 ↔ ExtrusionNutLockHNTR5-4:31
- Angle:48 (0 deg): FrameUpright:1 ↔ ExtrusionNutLockHNTR5-4:30
- Angle:49 (0 deg): FrameUpright:1 ↔ ExtrusionNutLockHNTR5-4:29
- Mate:390: FrameUpright:1 ↔ ExtrusionNutLockHNTR5-4:29
- Mate:391: FrameUpright:1 ↔ ExtrusionNutLockHNTR5-4:30
- Mate:392: FrameUpright:1 ↔ ExtrusionNutLockHNTR5-4:31
- Mate:393: FrameFrontBack:6 ↔ ExtrusionNutLockHNTR5-4:33
- Mate:394: FrameFrontBack:4 ↔ ExtrusionNutLockHNTR5-4:32
- Mate:395: FrameUpright:4 ↔ ExtrusionNutLockHNTR5-4:26
- Mate:396: FrameUpright:4 ↔ ExtrusionNutLockHNTR5-4:27
- Angle:50 (0 deg): FrameSide:4 ↔ ExtrusionNutLockHNTR5-4:19
- Angle:51 (0 deg): FrameSide:5 ↔ ExtrusionNutLockHNTR5-4:20
- Mate:397: FrameSide:4 ↔ ExtrusionNutLockHNTR5-4:19
- Mate:398: FrameSide:5 ↔ ExtrusionNutLockHNTR5-4:20
- Mate:399: FrameFrontBack:1 ↔ ExtrusionNutLockHNTR5-4:28
- Mate:424: PanelMount:6 ↔ ElectronicsLowerPanel:1
- Mate:425: PanelMount:1 ↔ ElectronicsLowerPanel:1
- Mate:426: PanelMount:5 ↔ ElectronicsLowerPanel:1
- Mate:427: PanelMount:2 ↔ ElectronicsLowerPanel:1
- Mate:429: PanelMount:4 ↔ ElectronicsLowerPanel:1
- Mate:430: FrameFrontBack:3 ↔ PanelMount:1
- Mate:431: FrameFrontBack:3 ↔ PanelMount:6
- Mate:432: FrameFrontBack:3 ↔ PanelMount:5
- Mate:433: FrameFrontBack:4 ↔ PanelMount:4
- Mate:435: FrameFrontBack:4 ↔ PanelMount:2
- Mate:436 (8.5 mm): FrameSide:3 ↔ PanelMount:2
- Mate:437 (8.5 mm): FrameSide:4 ↔ PanelMount:4
- Mate:438 (8.5 mm): FrameSide:4 ↔ PanelMount:1
- Mate:439 (8.5 mm): FrameSide:3 ↔ PanelMount:5
- Mate:440 (207.5 mm): FrameSide:3 ↔ PanelMount:6
- Mate:447: FrameFrontBack:5 ↔ PanelMount:11
- Mate:451: PanelMount:11 ↔ ElectronicsTopPanel:1
- Flush:138: FrameFrontBack:5 ↔ ElectronicsTopPanel:1
- Mate:460 (207.5 mm): FrameSide:6 ↔ PanelMount:11
- Mate:462: PanelMount:2 ↔ ElectronicsLowerPanel:1
- Mate:463: PanelMount:4 ↔ ElectronicsLowerPanel:1
- Mate:464: BoltWasher3x18:2 ↔ ElectronicsLowerPanel:1
- Mate:466: BoltWasher3x18:5 ↔ ElectronicsLowerPanel:1
- Mate:467: BoltWasher3x18:4 ↔ ElectronicsLowerPanel:1
- Mate:468: BoltWasher3x18:1 ↔ ElectronicsLowerPanel:1
- Mate:469: BoltWasher3x18:3 ↔ ElectronicsLowerPanel:1
- Mate:470: BoltWasher3x18:1 ↔ ElectronicsLowerPanel:1
- Mate:471: BoltWasher3x18:3 ↔ ElectronicsLowerPanel:1
- Mate:472: BoltWasher3x18:2 ↔ ElectronicsLowerPanel:1
- Mate:474: BoltWasher3x18:4 ↔ ElectronicsLowerPanel:1
- Mate:475: BoltWasher3x18:5 ↔ ElectronicsLowerPanel:1
- Mate:478: Nut3:3 ↔ BoltWasher3x18:5
- Mate:479: Nut3:3 ↔ PanelMount:4
- Angle:53 (0 deg): Nut3:3 ↔ PanelMount:4
- Mate:480: Nut3:1 ↔ BoltWasher3x18:2
- Angle:54 (0 deg): Nut3:1 ↔ PanelMount:2
- Mate:481: Nut3:1 ↔ PanelMount:2
- Mate:482: Nut3:2 ↔ BoltWasher3x18:4
- Mate:483: Nut3:2 ↔ PanelMount:1
- Angle:55 (0 deg): Nut3:2 ↔ PanelMount:1
- Mate:484: Nut3:4 ↔ BoltWasher3x18:1
- Mate:485: Nut3:4 ↔ PanelMount:6
- Angle:56 (0 deg): Nut3:4 ↔ PanelMount:6
- Mate:486: Nut3:5 ↔ BoltWasher3x18:3
- Mate:487: Nut3:5 ↔ PanelMount:5
- Angle:57 (0 deg): Nut3:5 ↔ PanelMount:5
- Mate:488: FrameFrontBack:5 ↔ PanelLedge:5
- Mate:489: FrameFrontBack:5 ↔ PanelLedge:4
- Mate:490: FrameFrontBack:6 ↔ PanelLedge:1
- Mate:492: FrameFrontBack:6 ↔ PanelLedge:3
- Mate:493: PanelLedge:1 ↔ ElectronicsTopPanel:1
- Mate:494: PanelLedge:3 ↔ ElectronicsTopPanel:1
- Mate:495: PanelLedge:5 ↔ ElectronicsTopPanel:1
- Mate:496: PanelLedge:4 ↔ ElectronicsTopPanel:1
- Mate:497 (8.5 mm): FrameSide:5 ↔ PanelLedge:5
- Mate:498 (8.5 mm): FrameSide:6 ↔ PanelLedge:4
- Mate:499 (8.5 mm): FrameSide:5 ↔ PanelLedge:3
- Mate:500 (8.5 mm): FrameSide:6 ↔ PanelLedge:1
- Mate:501: PanelMount:11 ↔ ElectronicsTopPanel:1
- Mate:502: ExtrusionNutHNKK5_4:1 ↔ SHCS4x10:8
- Angle:58 (0 deg): FrameFrontBack:6 ↔ ExtrusionNutHNKK5_4:1
- Mate:503: FrameFrontBack:6 ↔ ExtrusionNutHNKK5_4:1
- Mate:504: ExtrusionNutHNKK5_4:2 ↔ SHCS4x10:7
- Mate:505: FrameFrontBack:6 ↔ ExtrusionNutHNKK5_4:2
- Angle:59 (0 deg): FrameFrontBack:6 ↔ ExtrusionNutHNKK5_4:2
- Mate:506: ExtrusionNutHNKK5_4:3 ↔ SHCS4x10:2
- Angle:60 (0 deg): FrameFrontBack:6 ↔ ExtrusionNutHNKK5_4:3
- Mate:507: ExtrusionNutHNKK5_4:4 ↔ SHCS4x10:11
- Angle:61 (0 deg): FrameFrontBack:6 ↔ ExtrusionNutHNKK5_4:4
- Mate:508: FrameFrontBack:6 ↔ ExtrusionNutHNKK5_4:4
- Mate:509: FrameFrontBack:6 ↔ ExtrusionNutHNKK5_4:3
- Mate:510: ExtrusionNutHNKK5_4:6 ↔ SHCS4x10:10
- Mate:511: ExtrusionNutHNKK5_4:5 ↔ SHCS4x10:12
- Angle:62 (0 deg): FrameSide:6 ↔ ExtrusionNutHNKK5_4:5
- Angle:63 (0 deg): FrameSide:5 ↔ ExtrusionNutHNKK5_4:6
- Mate:512: FrameSide:5 ↔ ExtrusionNutHNKK5_4:6
- Mate:513: FrameSide:6 ↔ ExtrusionNutHNKK5_4:5
- Mate:514: ExtrusionNutHNKK5_4:7 ↔ SHCS4x10:4
- Mate:515: FrameUpright:3 ↔ ExtrusionNutHNKK5_4:7
- Angle:64 (0 deg): FrameUpright:3 ↔ ExtrusionNutHNKK5_4:7
- Mate:516: ExtrusionNutHNKK5_4:8 ↔ SHCS4x10:3
- Mate:517: FrameUpright:2 ↔ ExtrusionNutHNKK5_4:8
- Angle:65 (0 deg): FrameUpright:2 ↔ ExtrusionNutHNKK5_4:8
- Mate:518: ExtrusionNutHNKK5_4:9 ↔ SHCS4x10:5
- Mate:519: ExtrusionNutHNKK5_4:10 ↔ SHCS4x10:1
- Mate:520: ExtrusionNutHNKK5_4:12 ↔ SHCS4x10:9
- Mate:521: ExtrusionNutHNKK5_4:11 ↔ SHCS4x10:6
- Mate:522: FrameExtruderVerticalSupport:2 ↔ ExtrusionNutHNKK5_4:11
- Mate:523: FrameUpright:1 ↔ ExtrusionNutHNKK5_4:12
- Mate:524: FrameExtruderVerticalSupport:1 ↔ ExtrusionNutHNKK5_4:10
- Mate:525: FrameUpright:4 ↔ ExtrusionNutHNKK5_4:9
- Angle:66 (0 deg): FrameUpright:4 ↔ ExtrusionNutHNKK5_4:9
- Angle:67 (0 deg): FrameExtruderVerticalSupport:1 ↔ ExtrusionNutHNKK5_4:10
- Angle:68 (0 deg): FrameExtruderVerticalSupport:2 ↔ ExtrusionNutHNKK5_4:11
- Angle:69 (0 deg): FrameUpright:1 ↔ ExtrusionNutHNKK5_4:12
- Mate:538: EnclosurePanelLeft:1 ↔ SpoolHolderSingle:1
- Mate:539: EnclosurePanelRight:1 ↔ SpoolHolderSingle:2
- Mate:540: EnclosurePanelRight:1 ↔ SpoolHolderSingle:2
- Mate:541: EnclosurePanelRight:1 ↔ SpoolHolderSingle:2
- Mate:542: EnclosurePanelRight:1 ↔ SpoolHolderSingle:2
- Mate:543: EnclosurePanelLeft:1 ↔ SpoolHolderSingle:1
- Mate:544: EnclosurePanelLeft:1 ↔ SpoolHolderSingle:1
- Mate:545: EnclosurePanelLeft:1 ↔ SpoolHolderSingle:1
- Mate:546: EnclosurePanelLeft:1 ↔ FHS4x10:40
- Mate:547: EnclosurePanelLeft:1 ↔ FHS4x10:38
- Mate:548: EnclosurePanelLeft:1 ↔ FHS4x10:34
- Mate:549: EnclosurePanelLeft:1 ↔ FHS4x10:35
- Flush:143: EnclosurePanelLeft:1 ↔ FHS4x10:35
- Flush:144: EnclosurePanelLeft:1 ↔ FHS4x10:34
- Flush:145: EnclosurePanelLeft:1 ↔ FHS4x10:38
- Flush:146: EnclosurePanelLeft:1 ↔ FHS4x10:40
- Mate:550: EnclosurePanelRight:1 ↔ FHS4x10:36
- Mate:551: EnclosurePanelRight:1 ↔ FHS4x10:37
- Mate:552: EnclosurePanelRight:1 ↔ FHS4x10:41
- Mate:553: EnclosurePanelRight:1 ↔ FHS4x10:39
- Flush:147: EnclosurePanelRight:1 ↔ FHS4x10:39
- Flush:148: EnclosurePanelRight:1 ↔ FHS4x10:41
- Flush:149: EnclosurePanelRight:1 ↔ FHS4x10:37
- Flush:150: EnclosurePanelRight:1 ↔ FHS4x10:36
- Mate:554: Nut4:2 ↔ FHS4x10:41
- Mate:555: Nut4:4 ↔ FHS4x10:39
- Mate:556: Nut4:7 ↔ FHS4x10:36
- Mate:557: Nut4:5 ↔ FHS4x10:37
- Mate:558: Nut4:1 ↔ FHS4x10:38
- Mate:559: Nut4:3 ↔ FHS4x10:40
- Mate:560: Nut4:6 ↔ FHS4x10:34
- Mate:561: Nut4:8 ↔ FHS4x10:35
- Mate:562: Nut4:2 ↔ SpoolHolderSingle:2
- Mate:563: Nut4:7 ↔ SpoolHolderSingle:2
- Mate:564: Nut4:4 ↔ SpoolHolderSingle:2
- Mate:565: Nut4:5 ↔ SpoolHolderSingle:2
- Angle:73 (0 deg): Nut4:5 ↔ SpoolHolderSingle:2
- Angle:74 (0 deg): Nut4:4 ↔ SpoolHolderSingle:2
- Angle:75 (0 deg): Nut4:2 ↔ SpoolHolderSingle:2
- Angle:76 (0 deg): Nut4:7 ↔ SpoolHolderSingle:2
- Mate:566: Nut4:1 ↔ SpoolHolderSingle:1
- Mate:567: Nut4:3 ↔ SpoolHolderSingle:1
- Mate:568: Nut4:6 ↔ SpoolHolderSingle:1
- Mate:569: Nut4:8 ↔ SpoolHolderSingle:1
- Angle:77 (0 deg): Nut4:8 ↔ SpoolHolderSingle:1
- Angle:78 (0 deg): Nut4:6 ↔ SpoolHolderSingle:1
- Angle:79 (0 deg): Nut4:1 ↔ SpoolHolderSingle:1
- Angle:80 (0 deg): Nut4:3 ↔ SpoolHolderSingle:1
- Mate:570: FrameFrontBack:4 ↔ PanelLedge:6
- Flush:151 (3.237 mm): FrameFrontBack:4 ↔ PanelLedge:6
- Mate:571: PanelLedge:6 ↔ ElectronicsLowerPanel:1
- Mate:572: FHS4x10:47 ↔ PanelLedge:6
- Mate:573: FHS4x10:46 ↔ PanelMount:4
- Mate:574: FHS4x10:45 ↔ PanelLedge:5
- Mate:575: FHS4x10:44 ↔ PanelMount:11
- Mate:576: FHS4x10:43 ↔ PanelMount:2
- Mate:577: FHS4x10:42 ↔ PanelLedge:4
- Flush:152: FHS4x10:42 ↔ PanelLedge:4
- Flush:153: FHS4x10:44 ↔ PanelMount:11
- Flush:154: FHS4x10:45 ↔ PanelLedge:5
- Flush:155: FHS4x10:43 ↔ PanelMount:2
- Flush:156: FHS4x10:47 ↔ PanelLedge:6
- Flush:157: FHS4x10:46 ↔ PanelMount:4
- Flush:158: PanelLedge:6 ↔ PanelMount:6
- Mate:578: FHS4x10:48 ↔ PanelLedge:3
- Flush:159: FHS4x10:48 ↔ PanelLedge:3
- Mate:579: FHS4x10:49 ↔ PanelLedge:1
- Flush:160: FHS4x10:49 ↔ PanelLedge:1
- Mate:580: FHS4x10:50 ↔ PanelMount:1
- Flush:161: FHS4x10:50 ↔ PanelMount:1
- Mate:581: FHS4x10:51 ↔ PanelMount:6
- Flush:162: FHS4x10:51 ↔ PanelMount:6
- Mate:582: FHS4x10:52 ↔ PanelMount:5
- Flush:163: FHS4x10:52 ↔ PanelMount:5
- Mate:583: ExtrusionNutHNKK5_4:17 ↔ FHS4x10:43
- Mate:584: ExtrusionNutHNKK5_4:18 ↔ FHS4x10:47
- Mate:585: ExtrusionNutHNKK5_4:19 ↔ FHS4x10:46
- Mate:586: ExtrusionNutHNKK5_4:20 ↔ FHS4x10:50
- Mate:587: ExtrusionNutHNKK5_4:21 ↔ FHS4x10:51
- Mate:588: ExtrusionNutHNKK5_4:22 ↔ FHS4x10:52
- Mate:589: ExtrusionNutHNKK5_4:23 ↔ FHS4x10:42
- Mate:590: ExtrusionNutHNKK5_4:24 ↔ FHS4x10:44
- Mate:591: ExtrusionNutHNKK5_4:25 ↔ FHS4x10:45
- Mate:592: ExtrusionNutHNKK5_4:26 ↔ FHS4x10:48
- Mate:593: ExtrusionNutHNKK5_4:27 ↔ FHS4x10:49
- Angle:81 (0 deg): FrameFrontBack:6 ↔ ExtrusionNutHNKK5_4:26
- Angle:82 (0 deg): FrameFrontBack:6 ↔ ExtrusionNutHNKK5_4:27
- Angle:83 (0 deg): FrameFrontBack:3 ↔ ExtrusionNutHNKK5_4:22
- Angle:84 (0 deg): FrameFrontBack:3 ↔ ExtrusionNutHNKK5_4:21
- Angle:85 (0 deg): FrameFrontBack:3 ↔ ExtrusionNutHNKK5_4:20
- Angle:86 (0 deg): FrameFrontBack:5 ↔ ExtrusionNutHNKK5_4:25
- Angle:87 (0 deg): FrameFrontBack:5 ↔ ExtrusionNutHNKK5_4:24
- Angle:88 (0 deg): FrameFrontBack:5 ↔ ExtrusionNutHNKK5_4:23
- Angle:89 (0 deg): FrameFrontBack:4 ↔ ExtrusionNutHNKK5_4:17
- Angle:90 (0 deg): FrameFrontBack:4 ↔ ExtrusionNutHNKK5_4:18
- Angle:91 (0 deg): FrameFrontBack:4 ↔ ExtrusionNutHNKK5_4:19
- Mate:594: FrameFrontBack:6 ↔ ExtrusionNutHNKK5_4:26
- Mate:595: FrameFrontBack:4 ↔ ExtrusionNutHNKK5_4:19
- Mate:596: FrameFrontBack:3 ↔ ExtrusionNutHNKK5_4:20
- Mate:597: FrameFrontBack:3 ↔ ExtrusionNutHNKK5_4:24
- Mate:598: FrameFrontBack:3 ↔ ExtrusionNutHNKK5_4:21
- Mate:599: FrameFrontBack:3 ↔ ExtrusionNutHNKK5_4:22
- Mate:600: FrameFrontBack:5 ↔ ExtrusionNutHNKK5_4:23
- Mate:601: FrameFrontBack:4 ↔ ExtrusionNutHNKK5_4:18
- Mate:602: FrameFrontBack:4 ↔ ExtrusionNutHNKK5_4:17
- Mate:603: FrameFrontBack:6 ↔ ExtrusionNutHNKK5_4:27
- Mate:604: FrameFrontBack:5 ↔ ElectronicsTopPanel:1
- Mate:605: BoltWasher3x18:6 ↔ PanelMount:11
- Mate:606: BoltWasher3x18:6 ↔ ElectronicsTopPanel:1
- Mate:607: Nut3:6 ↔ BoltWasher3x18:6
- Mate:608: Nut3:6 ↔ PanelMount:11
- Angle:92 (0 deg): Nut3:6 ↔ PanelMount:11
- Angle:93 (0 deg): FrameSide:2 ↔ ExtrusionNutHNKK5_5:1
- Mate:609: FrameSide:2 ↔ ExtrusionNutHNKK5_5:1
- Mate:610: FrameSide:2 ↔ FrameHandle:1
- Flush:164: FrameSide:2 ↔ FrameHandle:1
- Mate:611: FrameHandle:1 ↔ ExtrusionNutHNKK5_5:1
- Angle:94 (0 deg): FrameSide:2 ↔ ExtrusionNutHNKK5_5:2
- Mate:612: FrameSide:2 ↔ ExtrusionNutHNKK5_5:2
- Mate:613: FrameHandle:1 ↔ ExtrusionNutHNKK5_5:2
- [Mate]: FrameHandle:2 ↔ ExtrusionNutHNKK5_5:3
- [Mate]: FrameHandle:2 ↔ ExtrusionNutHNKK5_5:4
- Angle:95 (0 deg): FrameSide:1 ↔ ExtrusionNutHNKK5_5:3
- Angle:96 (0 deg): FrameSide:1 ↔ ExtrusionNutHNKK5_5:4
- Mate:616: FrameSide:1 ↔ ExtrusionNutHNKK5_5:3
- Mate:617: FrameSide:1 ↔ ExtrusionNutHNKK5_5:4
- Flush:165: FrameSide:1 ↔ FrameHandle:2
- Mate:618: FrameSide:1 ↔ FrameHandle:2
## Named parameters: d167_d166 = 0 mm, d1049_d1045 = 0 mm, d1050_d1048 = 0 mm
